# Autodesk Inventor assembly: pmi
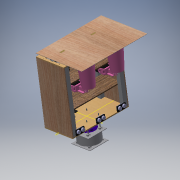
[picture p0: Inventor's stored thumbnail of the model, 180x180]
Saved by Autodesk Inventor 2019 (Build 230136000, 136)
## iProperties
Created: 2020-02-16
Part Number: pmi
Document SubType Name: Assembly
Designer: franc
Author: franc
## Documents named in this file (16)
- C:\Users\franc\Desktop\EsialRobotik\Mecanique\2020\pmi\pmi.iam
- C:\Users\franc\Desktop\EsialRobotik\Mecanique\2020\pmi\socle-robot.ipt
- C:\Users\franc\Desktop\EsialRobotik\Mecanique\base_roulante\base_roulante_pmi.iam
- C:\Users\franc\Desktop\EsialRobotik\Mecanique\composants\Profile\calle-pmi.iam
- C:\Users\franc\Desktop\EsialRobotik\Mecanique\2020\pmi\face-laterale.ipt
- C:\Users\franc\Desktop\EsialRobotik\Mecanique\2020\robot\support_arriere.iam
- C:\Users\franc\Desktop\EsialRobotik\Mecanique\2020\pmi\toit.iam
- C:\Users\franc\Desktop\EsialRobotik\Mecanique\composants\SRF04\SRF04_sur_support.iam
- C:\Users\franc\Desktop\EsialRobotik\Mecanique\2020\pmi\profile_alu.ipt
- C:\Users\franc\Desktop\EsialRobotik\Mecanique\composants\Profile\equerreEtage.ipt
- C:\Users\franc\Desktop\EsialRobotik\Mecanique\2020\pmi\etage.ipt
- C:\Users\franc\Desktop\EsialRobotik\Mecanique\base_roulante\sol.ipt
- C:\Users\franc\Desktop\EsialRobotik\Mecanique\2020\elements\bouees.ipt
- C:\Users\franc\Desktop\EsialRobotik\Mecanique\composants\AX12\AX12.iam
- C:\Users\franc\Desktop\EsialRobotik\Mecanique\composants\AX12\F3.ipt
- C:\Users\franc\Desktop\EsialRobotik\Mecanique\2020\pmi\bras.iam
## Components (33 placed, 15 different names)
1. socle-robot:1 — Placage:1, Placage:2, Placage:3, Placage:4, Placage:5, Placage:6, Placage:7, Affleurement:1, Affleurement:2, Affleurement:3, Affleurement:4, Affleurement:5, Affleurement:6, Affleurement:7, Affleurement:8, Placage:8, Affleurement:9, Affleurement:10, Placage:9, Affleurement:11, Affleurement:12, Placage:23, Placage:24, Placage:27, Placage:28, Placage:29, Placage:31, Placage:33, Placage:34, Placage:41, Placage:42, Affleurement:25, Affleurement:26
2. base_roulante_pmi:1 [sub-assembly] — Placage:1, Placage:2, Placage:3
3. calle-pmi:1 [sub-assembly] — Placage:4, Affleurement:2, Affleurement:3, Placage:43
4. calle-pmi:2 [sub-assembly] — Placage:5, Affleurement:1, Affleurement:4
5. calle-pmi:3 [sub-assembly] — Placage:6, Affleurement:5, Affleurement:6
6. calle-pmi:4 [sub-assembly] — Placage:7, Affleurement:7, Affleurement:8
7. face-laterale:1 — Placage:9, Affleurement:11, Affleurement:12, Affleurement:13, Affleurement:14, Affleurement:16, Placage:22, Affleurement:18, Placage:26, Affleurement:19, Placage:38, Placage:55
8. face-laterale:2 — Placage:8, Affleurement:9, Affleurement:10, Placage:11, Placage:12, Affleurement:15, Placage:21, Affleurement:17, Placage:25, Affleurement:20, Placage:40, Placage:53
9. support_arriere:1 [sub-assembly] — Placage:11, Affleurement:13, Affleurement:14
10. toit:1 [sub-assembly] — Placage:12, Affleurement:15, Affleurement:16, Placage:13, Placage:14, Placage:15, Placage:16, Placage:17, Placage:18, Placage:19, Placage:20
11. SRF04_sur_support:1 [sub-assembly] — Placage:13, Placage:14
12. SRF04_sur_support:2 [sub-assembly] — Placage:16, Placage:19
13. SRF04_sur_support:3 [sub-assembly] — Placage:17, Placage:18
14. SRF04_sur_support:4 [sub-assembly] — Placage:15, Placage:20
15. profile_alu:1 — Placage:22, Affleurement:18, Placage:24, Placage:35, Affleurement:23
16. profile_alu:2 — Placage:26, Affleurement:19, Placage:28, Placage:30, Affleurement:21, Placage:39
17. profile_alu:3 — Placage:25, Affleurement:20, Placage:27, Placage:32, Affleurement:22, Placage:37
18. profile_alu:4 — Placage:21, Affleurement:17, Placage:23, Placage:36, Affleurement:24
19. equerreEtage:1 — Placage:31, Placage:32, Affleurement:22
20. equerreEtage:2 — Placage:29, Placage:30, Affleurement:21
21. equerreEtage:3 — Placage:34, Placage:35, Affleurement:23
22. equerreEtage:4 — Placage:33, Placage:36, Affleurement:24
23. etage:1 — Placage:39, Placage:40, Placage:42
24. etage:2 — Placage:37, Placage:38, Placage:41, Placage:49, Affleurement:27, Placage:50, Affleurement:28
25. sol:1 — Placage:43, Affleurement:25, Affleurement:26, Placage:44, Placage:45
26. bouees:1 — Placage:44
27. bouees:2 — Placage:45
28. AX12:1 [sub-assembly] — Placage:51, Placage:52, Placage:54, Affleurement:28, Placage:58, Placage:59
29. AX12:2 [sub-assembly] — Placage:46, Placage:47, Placage:48, Affleurement:27, Placage:56, Placage:57
30. F3:1 — Placage:50, Placage:51, Placage:52, Placage:54, Placage:55
31. F3:2 — Placage:46, Placage:47, Placage:48, Placage:49, Placage:53
32. bras:1 [sub-assembly] — Placage:58, Placage:59
33. bras:2 [sub-assembly] — Placage:56, Placage:57
## Relationships (86: Mate 58, Flush 28)
- Placage:1 [Mate]: socle-robot:1 ↔ base_roulante_pmi:1
- Placage:2 [Mate]: socle-robot:1 ↔ base_roulante_pmi:1
- Placage:3 [Mate]: socle-robot:1 ↔ base_roulante_pmi:1
- Placage:4 [Mate]: socle-robot:1 ↔ calle-pmi:1
- Placage:5 [Mate]: socle-robot:1 ↔ calle-pmi:2
- Placage:6 [Mate]: socle-robot:1 ↔ calle-pmi:3
- Placage:7 [Mate]: socle-robot:1 ↔ calle-pmi:4
- Affleurement:1 [Flush]: socle-robot:1 ↔ calle-pmi:2
- Affleurement:2 [Flush]: socle-robot:1 ↔ calle-pmi:1
- Affleurement:3 [Flush] (40 mm): socle-robot:1 ↔ calle-pmi:1
- Affleurement:4 [Flush] (40 mm): socle-robot:1 ↔ calle-pmi:2
- Affleurement:5 [Flush]: socle-robot:1 ↔ calle-pmi:3
- Affleurement:6 [Flush] (40 mm): socle-robot:1 ↔ calle-pmi:3
- Affleurement:7 [Flush]: socle-robot:1 ↔ calle-pmi:4
- Affleurement:8 [Flush] (40 mm): socle-robot:1 ↔ calle-pmi:4
- Placage:8 [Mate]: socle-robot:1 ↔ face-laterale:2
- Affleurement:9 [Flush]: socle-robot:1 ↔ face-laterale:2
- Affleurement:10 [Flush]: socle-robot:1 ↔ face-laterale:2
- Placage:9 [Mate]: socle-robot:1 ↔ face-laterale:1
- Affleurement:11 [Flush]: socle-robot:1 ↔ face-laterale:1
- Affleurement:12 [Flush]: socle-robot:1 ↔ face-laterale:1
- Placage:11 [Mate]: face-laterale:2 ↔ support_arriere:1
- Affleurement:13 [Flush]: face-laterale:1 ↔ support_arriere:1
- Affleurement:14 [Flush] (-30 mm): face-laterale:1 ↔ support_arriere:1
- Placage:12 [Mate]: face-laterale:2 ↔ toit:1
- Affleurement:15 [Flush]: face-laterale:2 ↔ toit:1
- Affleurement:16 [Flush]: face-laterale:1 ↔ toit:1
- Placage:13 [Mate]: toit:1 ↔ SRF04_sur_support:1
- Placage:14 [Mate]: toit:1 ↔ SRF04_sur_support:1
- Placage:15 [Mate]: toit:1 ↔ SRF04_sur_support:4
- Placage:16 [Mate]: toit:1 ↔ SRF04_sur_support:2
- Placage:17 [Mate]: toit:1 ↔ SRF04_sur_support:3
- Placage:18 [Mate]: toit:1 ↔ SRF04_sur_support:3
- Placage:19 [Mate]: toit:1 ↔ SRF04_sur_support:2
- Placage:20 [Mate]: toit:1 ↔ SRF04_sur_support:4
- Placage:21 [Mate]: face-laterale:2 ↔ profile_alu:4
- Affleurement:17 [Flush]: face-laterale:2 ↔ profile_alu:4
- Placage:22 [Mate]: face-laterale:1 ↔ profile_alu:1
- Affleurement:18 [Flush]: face-laterale:1 ↔ profile_alu:1
- Placage:23 [Mate]: socle-robot:1 ↔ profile_alu:4
- Placage:24 [Mate]: socle-robot:1 ↔ profile_alu:1
- Placage:25 [Mate]: face-laterale:2 ↔ profile_alu:3
- Placage:26 [Mate]: face-laterale:1 ↔ profile_alu:2
- Affleurement:19 [Flush] (5 mm): face-laterale:1 ↔ profile_alu:2
- Affleurement:20 [Flush] (5 mm): face-laterale:2 ↔ profile_alu:3
- Placage:27 [Mate]: socle-robot:1 ↔ profile_alu:3
- Placage:28 [Mate]: socle-robot:1 ↔ profile_alu:2
- Placage:29 [Mate]: socle-robot:1 ↔ equerreEtage:2
- Placage:30 [Mate]: profile_alu:2 ↔ equerreEtage:2
- Affleurement:21 [Flush]: profile_alu:2 ↔ equerreEtage:2
- Placage:31 [Mate]: socle-robot:1 ↔ equerreEtage:1
- Placage:32 [Mate]: profile_alu:3 ↔ equerreEtage:1
- Affleurement:22 [Flush]: profile_alu:3 ↔ equerreEtage:1
- Placage:33 [Mate]: socle-robot:1 ↔ equerreEtage:4
- Placage:34 [Mate]: socle-robot:1 ↔ equerreEtage:3
- Placage:35 [Mate]: profile_alu:1 ↔ equerreEtage:3
- Affleurement:23 [Flush]: profile_alu:1 ↔ equerreEtage:3
- Placage:36 [Mate]: profile_alu:4 ↔ equerreEtage:4
- Affleurement:24 [Flush]: profile_alu:4 ↔ equerreEtage:4
- Placage:37 [Mate]: profile_alu:3 ↔ etage:2
- Placage:38 [Mate]: face-laterale:1 ↔ etage:2
- Placage:39 [Mate]: profile_alu:2 ↔ etage:1
- Placage:40 [Mate]: face-laterale:2 ↔ etage:1
- Placage:41 [Mate] (90 mm): socle-robot:1 ↔ etage:2
- Placage:42 [Mate] (200 mm): socle-robot:1 ↔ etage:1
- Placage:43 [Mate]: calle-pmi:1 ↔ sol:1
- Affleurement:25 [Flush]: socle-robot:1 ↔ sol:1
- Affleurement:26 [Flush]: socle-robot:1 ↔ sol:1
- Placage:44 [Mate]: sol:1 ↔ bouees:1
- Placage:45 [Mate]: sol:1 ↔ bouees:2
- Placage:46 [Mate]: AX12:2 ↔ F3:2
- Placage:47 [Mate]: AX12:2 ↔ F3:2
- Placage:48 [Mate]: AX12:2 ↔ F3:2
- Placage:49 [Mate]: etage:2 ↔ F3:2
- Affleurement:27 [Flush]: etage:2 ↔ AX12:2
- Placage:50 [Mate]: etage:2 ↔ F3:1
- Placage:51 [Mate]: AX12:1 ↔ F3:1
- Placage:52 [Mate]: AX12:1 ↔ F3:1
- Placage:53 [Mate] (50 mm): face-laterale:2 ↔ F3:2
- Placage:54 [Mate]: AX12:1 ↔ F3:1
- Affleurement:28 [Flush]: etage:2 ↔ AX12:1
- Placage:55 [Mate] (50 mm): face-laterale:1 ↔ F3:1
- Placage:56 [Mate]: AX12:2 ↔ bras:2
- Placage:57 [Mate]: AX12:2 ↔ bras:2
- Placage:58 [Mate]: AX12:1 ↔ bras:1
- Placage:59 [Mate]: AX12:1 ↔ bras:1
